# Autodesk Inventor assembly: Hand cleaner station assembly
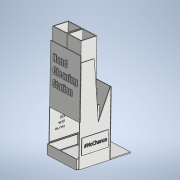
[picture p0: Inventor's stored thumbnail of the model, 180x180]
Saved by Autodesk Inventor 2020.2 (Build 242310000, 310)
## iProperties
Created: 2020-04-01
Part Number: Hand cleaner station assembly
Document SubType Name: Assembly
Designer: iamin
Author: iamin
## Documents named in this file (9)
- C:\Users\iamin\Documents\Modelling\hand cleaning station\Hand cleaner station assembly.iam
- C:\Users\iamin\Documents\Modelling\hand cleaning station\hand-cleaning-body.ipt
- C:\Users\iamin\Documents\Modelling\hand cleaning station\connector.ipt
- C:\Users\iamin\Documents\Modelling\hand cleaning station\soapy-water-tank.ipt
- C:\Users\iamin\Documents\Modelling\hand cleaning station\L-faucet.ipt
- C:\Users\iamin\Documents\Modelling\hand cleaning station\L-turning-knob.ipt
- C:\Users\iamin\Documents\Modelling\hand cleaning station\R-faucet.ipt
- C:\Users\iamin\Documents\Modelling\hand cleaning station\R-turning-knob.ipt
- C:\Users\iamin\Documents\Modelling\hand cleaning station\soap-collector-tray.ipt
## Components (10 placed, 8 different names)
1. hand-cleaning-body:1 — Mate:5, Mate:6, Mate:7, Mate:8, Mate:9, Mate:10, Mate:11, Mate:12, Mate:13, Mate:14, Mate:23, Mate:24
2. connector:1 — Mate:7, Mate:8, Mate:21, Mate:22
3. connector:2 — Mate:5, Mate:6, Mate:17, Mate:18
4. soapy-water-tank:1 — Mate:9, Mate:12, Mate:14
5. soapy-water-tank:2 — Mate:10, Mate:11, Mate:13
6. L-faucet:1 — Mate:15, Mate:16, Mate:17, Mate:18
7. L-turning-knob:1 — Mate:15, Mate:16
8. R-faucet:1 — Mate:19, Mate:20, Mate:21, Mate:22
9. R-turning-knob:1 — Mate:19, Mate:20
10. soap-collector-tray:1 — Mate:23, Mate:24
## Relationships (20: Mate 20)
- Mate:5: hand-cleaning-body:1 ↔ connector:2
- Mate:6: hand-cleaning-body:1 ↔ connector:2
- Mate:7: hand-cleaning-body:1 ↔ connector:1
- Mate:8: hand-cleaning-body:1 ↔ connector:1
- Mate:9: hand-cleaning-body:1 ↔ soapy-water-tank:1
- Mate:10: hand-cleaning-body:1 ↔ soapy-water-tank:2
- Mate:11: hand-cleaning-body:1 ↔ soapy-water-tank:2
- Mate:12: hand-cleaning-body:1 ↔ soapy-water-tank:1
- Mate:13: hand-cleaning-body:1 ↔ soapy-water-tank:2
- Mate:14: hand-cleaning-body:1 ↔ soapy-water-tank:1
- Mate:15: L-faucet:1 ↔ L-turning-knob:1
- Mate:16: L-faucet:1 ↔ L-turning-knob:1
- Mate:17: connector:2 ↔ L-faucet:1
- Mate:18: connector:2 ↔ L-faucet:1
- Mate:19: R-faucet:1 ↔ R-turning-knob:1
- Mate:20: R-faucet:1 ↔ R-turning-knob:1
- Mate:21: connector:1 ↔ R-faucet:1
- Mate:22: connector:1 ↔ R-faucet:1
- Mate:23: hand-cleaning-body:1 ↔ soap-collector-tray:1
- Mate:24: hand-cleaning-body:1 ↔ soap-collector-tray:1
